# Autodesk Inventor assembly: Base Chassis Assembly
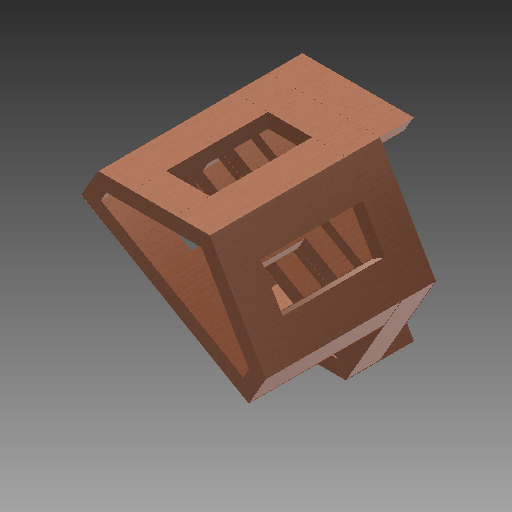
[picture p0: Inventor's stored thumbnail of the model, 512x512]
Saved by Autodesk Inventor 2017 (Build 210142000, 142)
## iProperties
Created: 2018-10-18
Part Number: Base Chassis Assembly
Document SubType Name: Assembly
Designer: Dell
Author: Dell
## Documents named in this file (6)
- C:\Users\Dell\Documents\GitHub\tr2\Base\Base Chassis Assembly.iam
- C:\Users\Dell\Documents\GitHub\tr2\BA01.ipt
- C:\Users\Dell\Documents\GitHub\tr2\BA02.ipt
- C:\Users\Dell\Documents\GitHub\tr2\Base\BA07.ipt
- C:\Users\Dell\Documents\GitHub\tr2\Base\BA08.ipt
- C:\Users\Dell\Documents\GitHub\tr2\Base\BA11.ipt
## Components (23 placed, 5 different names)
1. BA01:1
2. BA01:2
3. BA01:3
4. BA01:4
5. BA01:5
6. BA01:6
7. BA02:1
8. BA02:2
9. BA01:7
10. BA01:8
11. BA01:9
12. BA02:3
13. BA07:1
14. BA07:2
15. BA07:3
16. BA07:4
17. BA07:5
18. BA07:6
19. BA02:4
20. BA08:1
21. BA08:2
22. BA11:1
23. BA02:5
## Relationships (67: Mate 44, Flush 23)
- [Mate]: BA01:1 ↔ BA01:6
- [Mate]: BA01:2 ↔ BA01:6
- [Mate]: BA01:2 ↔ BA01:6
- [Mate]: BA01:2 ↔ BA01:6
- [Flush]: BA01:1 ↔ BA01:6
- [Mate]: BA01:1 ↔ BA01:6
- [Mate]: BA01:2 ↔ BA01:3
- [Mate]: BA01:2 ↔ BA01:3
- [Flush]: BA01:2 ↔ BA01:3
- [Mate]: BA01:1 ↔ BA01:5
- [Flush]: BA01:1 ↔ BA01:5
- [Mate]: BA01:1 ↔ BA01:5
- [Mate]: BA01:4 ↔ BA01:5
- [Flush]: BA01:4 ↔ BA01:5
- [Mate]: BA01:4 ↔ BA01:5
- [Mate]: BA01:5 ↔ BA02:1
- [Flush]: BA01:5 ↔ BA02:1
- [Mate]: BA01:5 ↔ BA02:1
- [Flush]: BA01:5 ↔ BA02:2
- [Mate]: BA01:5 ↔ BA02:2
- [Mate]: BA01:3 ↔ BA01:7
- [Mate]: BA01:3 ↔ BA01:7
- [Mate]: BA01:2 ↔ BA01:7
- [Flush]: BA01:6 ↔ BA01:8
- [Mate]: BA01:2 ↔ BA01:8
- [Mate]: BA01:6 ↔ BA01:8
- [Mate]: BA01:6 ↔ BA01:8
- [Mate]: BA01:8 ↔ BA01:9
- [Mate]: BA01:5 ↔ BA01:9
- [Mate]: BA01:1 ↔ BA01:9
- [Mate]: BA01:4 ↔ BA07:1
- [Flush]: BA01:4 ↔ BA07:1
- [Mate]: BA01:4 ↔ BA07:1
- [Mate]: BA07:1 ↔ BA07:2
- [Flush]: BA07:1 ↔ BA07:2
- [Flush]: BA01:3 ↔ BA07:2
- [Mate]: BA01:4 ↔ BA07:3
- [Flush]: BA07:1 ↔ BA07:3
- [Mate]: BA01:5 ↔ BA07:3
- [Mate]: BA07:3 ↔ BA07:4
- [Mate]: BA07:5 ↔ BA07:6
- [Mate]: BA07:5 ↔ BA07:6
- [Flush]: BA07:5 ↔ BA07:6
- [Mate]: BA01:2 ↔ BA07:6
- [Mate]: BA01:3 ↔ BA07:6
- [Flush]: BA01:7 ↔ BA07:6
- [Mate]: BA07:2 ↔ BA08:1
- [Flush]: BA07:2 ↔ BA08:1
- [Flush]: BA07:2 ↔ BA08:1
- [Mate]: BA07:1 ↔ BA08:2
- [Flush]: BA07:1 ↔ BA08:2
- [Flush]: BA07:1 ↔ BA08:2
- [Mate]: BA02:3 ↔ BA07:5
- [Mate]: BA07:3 ↔ BA07:4
- [Mate]: BA01:5 ↔ BA07:4
- [Flush]: BA02:3 ↔ BA07:5
- [Flush]: BA02:3 ↔ BA07:5
- [Flush]: BA07:5 ↔ BA02:4
- [Mate]: BA07:4 ↔ BA02:4
- [Mate]: BA01:5 ↔ BA02:2
- [Flush] (-44.45 mm): BA01:2 ↔ BA02:4
- [Mate]: BA02:4 ↔ BA11:1
- [Flush]: BA02:4 ↔ BA11:1
- [Mate] (171.45 mm): BA07:4 ↔ BA11:1
- [Mate]: BA01:2 ↔ BA02:5
- [Flush]: BA01:2 ↔ BA02:5
- [Mate] (63.5 mm): BA02:2 ↔ BA02:5
## Named parameters: d116_d113 = 0 mm
